# Autodesk Inventor assembly: 足ユニット
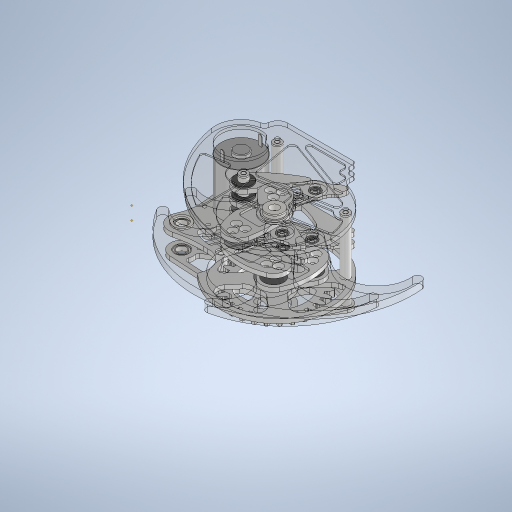
[picture p0: Inventor's stored thumbnail of the model, 512x512]
Saved by Autodesk Inventor 2023 (Build 270158000, 158)
## iProperties
Created: 2022-01-10
Part Number: 足ユニット
Document SubType Name: Assembly
Designer: acps
Author: acps
## Documents named in this file (20)
- C:\Users\acps\Documents\srdc\srdc_ksh\脚\足ユニット.iam
- C:\Users\acps\Documents\srdc\srdc_ksh\脚\足外フレーム.ipt
- C:\Users\acps\Documents\srdc\srdc_ksh\脚\足内フレーム.ipt
- C:\Users\acps\Documents\srdc\srdc_ksh\スペーサ\l40.ipt
- C:\Users\acps\Documents\srdc\srdc_ksh\カム\カム4.ipt
- C:\Users\acps\Documents\srdc\srdc_ksh\オイレス\w5f15-17n.ipt
- C:\Users\acps\Documents\srdc\srdc_ksh\モータ\M-RS-380.ipt
- C:\Users\acps\Documents\srdc\srdc_ksh\脚\モータマウント.ipt
- C:\Users\acps\Documents\srdc\srdc_ksh\ベアリング\φ6φ12ベアリングa.ipt
- C:\Users\acps\Documents\srdc\srdc_ksh\脚\ギア\初段_多段ギア.iam
- C:\Users\acps\Documents\srdc\srdc_ksh\脚\ギア\ぴにょん.ipt
- C:\Users\acps\Documents\srdc\srdc_ksh\ベアリング\M-φ4φ8a.ipt
- C:\Users\acps\Documents\srdc\srdc_ksh\ピン\φ4ピン　L20.ipt
- C:\Users\acps\Documents\srdc\srdc_ksh\ベアリング\φ4φ8ベアリングa.ipt
- C:\Users\acps\Documents\srdc\srdc_ksh\脚\ギア\最終段m2z28t4.ipt
- C:\Users\acps\Documents\srdc\srdc_ksh\脚\クランク.iam
- C:\Users\acps\Documents\srdc\srdc_ksh\脚\揺動節+ヘッケン.iam
- C:\Users\acps\Documents\srdc\srdc_ksh\スペーサ\l14.ipt
- C:\Users\acps\Documents\srdc\srdc_ksh\脚\ギア抑え.ipt
- C:\Users\acps\Documents\srdc\srdc_ksh\ベアリング\φ6φ10ベアリングa.ipt
## Components (27 placed, 19 different names)
1. l40:1 — Insert:68, Mate:72
2. l40:2 — Insert:67
3. l40:3 — Mate:49, Mate:51, Mate:53, Mate:55, Mate:64, Insert:65
4. カム4:1 — Insert:9, Insert:51, Mate:68, Mate:69, Mate:70, Insert:75
5. w5f15-17n:1 — Insert:9
6. M-RS-380:1 — Insert:31, Mate:38, Insert:32, Mate:61, Mate:62, Mate:71
7. φ6φ12ベアリングa:1 — Insert:86
8. モータマウント:1 — Insert:31, Mate:61, Mate:71, Insert:83, Mate:76
9. ぴにょん:1 — Mate:38, Insert:32
10. M-φ4φ8a:1 — Mate:41, Mate:42, Insert:80, Insert:81
11. 初段_多段ギア:1 [sub-assembly] — Mate:41, Mate:62
12. φ4ピン　L20:1 — Mate:42, Insert:81
13. φ4φ8ベアリングa:1
14. 最終段m2z28t4:1 — Mate:69, Mate:70, Insert:75
15. クランク:1 [sub-assembly] — Insert:51, Mate:50, Insert:52, Mate:52, Insert:54, Mate:54, Insert:55, Mate:56, Insert:56, Mate:68
16. 揺動節+ヘッケン:1 [sub-assembly] — Mate:51, Mate:52, Insert:54
17. 揺動節+ヘッケン:2 [sub-assembly] — Mate:53, Mate:54, Insert:55
18. 揺動節+ヘッケン:3 [sub-assembly] — Mate:55, Mate:56, Insert:56
19. 揺動節+ヘッケン:4 [sub-assembly] — Mate:49, Mate:50, Insert:52
20. l14:1
21. l14:2 — Insert:79, Insert:82
22. l14:3
23. 足外フレーム:1 — Mate:64, Insert:65, Insert:67, Insert:68, Mate:74, Mate:75, Insert:86
24. ギア抑え:1 — Insert:79, Mate:72, Insert:80, Insert:84
25. 足内フレーム:1 — Mate:74, Mate:75, Insert:82, Insert:83, Mate:76, Insert:85
26. φ6φ10ベアリングa:1 — Insert:84
27. φ6φ10ベアリングa:2 — Insert:85
## Relationships (42: Mate 22, Insert 20)
- Insert:9: カム4:1 ↔ w5f15-17n:1
- Insert:31: M-RS-380:1 ↔ モータマウント:1
- Mate:38: M-RS-380:1 ↔ ぴにょん:1
- Insert:32: M-RS-380:1 ↔ ぴにょん:1
- Mate:41: M-φ4φ8a:1 ↔ 初段_多段ギア:1
- Mate:42: M-φ4φ8a:1 ↔ φ4ピン　L20:1
- Insert:51: カム4:1 ↔ クランク:1
- Mate:49: l40:3 ↔ 揺動節+ヘッケン:4
- Mate:50: クランク:1 ↔ 揺動節+ヘッケン:4
- Insert:52 (0.25 mm): クランク:1 ↔ 揺動節+ヘッケン:4
- Mate:51: l40:3 ↔ 揺動節+ヘッケン:1
- Mate:52: クランク:1 ↔ 揺動節+ヘッケン:1
- Insert:54 (0.25 mm): クランク:1 ↔ 揺動節+ヘッケン:1
- Mate:53: l40:3 ↔ 揺動節+ヘッケン:2
- Mate:54: クランク:1 ↔ 揺動節+ヘッケン:2
- Insert:55 (0.25 mm): クランク:1 ↔ 揺動節+ヘッケン:2
- Mate:55: l40:3 ↔ 揺動節+ヘッケン:3
- Mate:56: クランク:1 ↔ 揺動節+ヘッケン:3
- Insert:56 (0.25 mm): クランク:1 ↔ 揺動節+ヘッケン:3
- Mate:61: M-RS-380:1 ↔ モータマウント:1
- Mate:62 (0.3 mm): M-RS-380:1 ↔ 初段_多段ギア:1
- Mate:64: l40:3 ↔ 足外フレーム:1
- Insert:65: l40:3 ↔ 足外フレーム:1
- Insert:67: l40:2 ↔ 足外フレーム:1
- Insert:68: l40:1 ↔ 足外フレーム:1
- Mate:68: カム4:1 ↔ クランク:1
- Mate:69: カム4:1 ↔ 最終段m2z28t4:1
- Mate:70: カム4:1 ↔ 最終段m2z28t4:1
- Insert:75: カム4:1 ↔ 最終段m2z28t4:1
- Mate:71: M-RS-380:1 ↔ モータマウント:1
- Insert:79: l14:2 ↔ ギア抑え:1
- Mate:72: l40:1 ↔ ギア抑え:1
- Insert:80: M-φ4φ8a:1 ↔ ギア抑え:1
- Insert:81 (0.5 mm): M-φ4φ8a:1 ↔ φ4ピン　L20:1
- Mate:74: 足外フレーム:1 ↔ 足内フレーム:1
- Mate:75: 足外フレーム:1 ↔ 足内フレーム:1
- Insert:82: l14:2 ↔ 足内フレーム:1
- Insert:83: モータマウント:1 ↔ 足内フレーム:1
- Mate:76: モータマウント:1 ↔ 足内フレーム:1
- Insert:84: ギア抑え:1 ↔ φ6φ10ベアリングa:1
- Insert:85: 足内フレーム:1 ↔ φ6φ10ベアリングa:2
- Insert:86: φ6φ12ベアリングa:1 ↔ 足外フレーム:1
